# Autodesk Inventor assembly: Under Track Arms
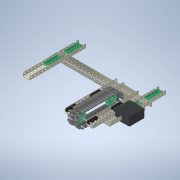
[picture p0: Inventor's stored thumbnail of the model, 180x180]
Saved by Autodesk Inventor 2020 (Build 240168000, 168)
## iProperties
Created: 2019-09-15
Part Number: Under Track Arms
Document SubType Name: Assembly
Designer: Corey
Author: Corey
## Documents named in this file (6)
- C:\Users\Corey\Documents\Tower-Takeover-CAD\Parts\Under Track Arms.iam
- C:\Users\Corey\Documents\Tower-Takeover-CAD\Parts\Structure\C-Channels\Aluminum\2-Wide\Aluminum C-Channel 1x2x1x16.ipt
- C:\Users\Corey\Documents\Tower-Takeover-CAD\Parts\Motion\Inner Acetal Slide Truck.ipt
- C:\Users\Corey\Documents\Tower-Takeover-CAD\Parts\Structure\C-Channels\Aluminum\2-Wide\Aluminum C-Channel 1x2x1x25.ipt
- C:\Users\Corey\Documents\Tower-Takeover-CAD\Parts\Motion\Washers & Spacers\Spacer (Nylon), 0.125''.ipt
- C:\Users\Corey\Documents\Tower-Takeover-CAD\Parts\Right Side Arm Intake.iam
## Components (16 placed, 5 different names)
1. Aluminum C-Channel 1x2x1x16:1 — Insert:61, Insert:62, Insert:63, Insert:64, Mate:46, Flush:7, Flush:8
2. Aluminum C-Channel 1x2x1x16:2 — Insert:67, Insert:68, Insert:69, Insert:70, Flush:5, Mate:45, Flush:6
3. Inner Acetal Slide Truck:1 — Mate:43, Insert:71, Insert:72
4. Inner Acetal Slide Truck:2 — Mate:44, Insert:73, Insert:74
5. Inner Acetal Slide Truck:3 — Mate:40, Mate:41, Mate:42
6. Inner Acetal Slide Truck:4 — Mate:39, Insert:65, Insert:66
7. Aluminum C-Channel 1x2x1x25:1 — Flush:5, Mate:45, Flush:6, Mate:46, Flush:7, Flush:8, Mate:47, Flush:9, Flush:10
8. Spacer (Nylon), 0.125'':1 — Insert:61, Mate:39, Insert:65
9. Spacer (Nylon), 0.125'':2 — Insert:62, Insert:66
10. Spacer (Nylon), 0.125'':3 — Insert:63, Mate:40, Mate:41
11. Spacer (Nylon), 0.125'':4 — Insert:64, Mate:42
12. Spacer (Nylon), 0.125'':5 — Insert:67, Mate:43, Insert:72
13. Spacer (Nylon), 0.125'':6 — Insert:68, Insert:71
14. Spacer (Nylon), 0.125'':7 — Insert:69, Mate:44, Insert:74
15. Spacer (Nylon), 0.125'':8 — Insert:70, Insert:73
16. Right Side Arm Intake:1 [sub-assembly] — Mate:47, Flush:9, Flush:10
## Relationships (29: Insert 14, Mate 9, Flush 6)
- Insert:61: Aluminum C-Channel 1x2x1x16:1 ↔ Spacer (Nylon), 0.125'':1
- Insert:62: Aluminum C-Channel 1x2x1x16:1 ↔ Spacer (Nylon), 0.125'':2
- Insert:63: Aluminum C-Channel 1x2x1x16:1 ↔ Spacer (Nylon), 0.125'':3
- Insert:64: Aluminum C-Channel 1x2x1x16:1 ↔ Spacer (Nylon), 0.125'':4
- Mate:39: Inner Acetal Slide Truck:4 ↔ Spacer (Nylon), 0.125'':1
- Mate:40: Inner Acetal Slide Truck:3 ↔ Spacer (Nylon), 0.125'':3
- Insert:65: Inner Acetal Slide Truck:4 ↔ Spacer (Nylon), 0.125'':1
- Insert:66: Inner Acetal Slide Truck:4 ↔ Spacer (Nylon), 0.125'':2
- Mate:41: Inner Acetal Slide Truck:3 ↔ Spacer (Nylon), 0.125'':3
- Mate:42: Inner Acetal Slide Truck:3 ↔ Spacer (Nylon), 0.125'':4
- Insert:67: Aluminum C-Channel 1x2x1x16:2 ↔ Spacer (Nylon), 0.125'':5
- Insert:68: Aluminum C-Channel 1x2x1x16:2 ↔ Spacer (Nylon), 0.125'':6
- Insert:69: Aluminum C-Channel 1x2x1x16:2 ↔ Spacer (Nylon), 0.125'':7
- Insert:70: Aluminum C-Channel 1x2x1x16:2 ↔ Spacer (Nylon), 0.125'':8
- Mate:43: Inner Acetal Slide Truck:1 ↔ Spacer (Nylon), 0.125'':5
- Insert:71: Inner Acetal Slide Truck:1 ↔ Spacer (Nylon), 0.125'':6
- Insert:72: Inner Acetal Slide Truck:1 ↔ Spacer (Nylon), 0.125'':5
- Mate:44: Inner Acetal Slide Truck:2 ↔ Spacer (Nylon), 0.125'':7
- Insert:73: Inner Acetal Slide Truck:2 ↔ Spacer (Nylon), 0.125'':8
- Insert:74: Inner Acetal Slide Truck:2 ↔ Spacer (Nylon), 0.125'':7
- Flush:5: Aluminum C-Channel 1x2x1x16:2 ↔ Aluminum C-Channel 1x2x1x25:1
- Mate:45: Aluminum C-Channel 1x2x1x16:2 ↔ Aluminum C-Channel 1x2x1x25:1
- Flush:6: Aluminum C-Channel 1x2x1x16:2 ↔ Aluminum C-Channel 1x2x1x25:1
- Mate:46: Aluminum C-Channel 1x2x1x16:1 ↔ Aluminum C-Channel 1x2x1x25:1
- Flush:7: Aluminum C-Channel 1x2x1x16:1 ↔ Aluminum C-Channel 1x2x1x25:1
- Flush:8: Aluminum C-Channel 1x2x1x16:1 ↔ Aluminum C-Channel 1x2x1x25:1
- Mate:47: Aluminum C-Channel 1x2x1x25:1 ↔ Right Side Arm Intake:1
- Flush:9: Aluminum C-Channel 1x2x1x25:1 ↔ Right Side Arm Intake:1
- Flush:10: Aluminum C-Channel 1x2x1x25:1 ↔ Right Side Arm Intake:1
